# Autodesk Inventor assembly: fox
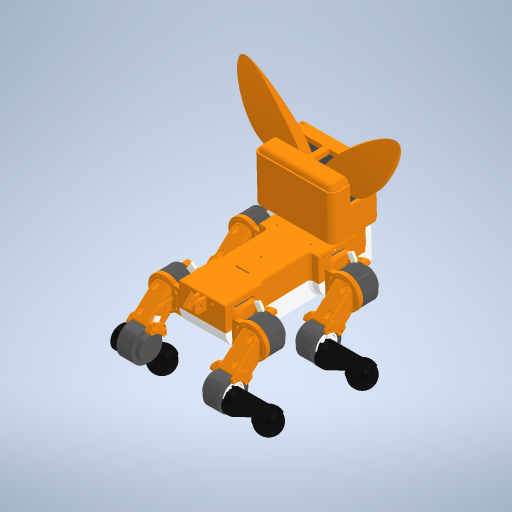
[picture p0: Inventor's stored thumbnail of the model, 512x512]
Saved by Autodesk Inventor 2024.2 (Build 282272000, 272)
## iProperties
Created: 2025-09-19
Part Number: fox
Document SubType Name: Assembly
Designer: AdminForWorker
Title: Pupper v3.5 v16
Author: AdminForWorker
## Documents named in this file (11)
- D:\dog\fox\construction\fox\fox.iam
- D:\dog\fox\construction\fox\legs\Lower leg - Short Short V6 (No Pinch) v20.iam
- D:\dog\fox\construction\fox\legs\Lower leg - Short Short V6 (No Pinch) v20_1.iam
- D:\dog\fox\construction\fox\legs\две части ног.iam
- D:\dog\fox\construction\fox\body\тело лисы.iam
- D:\dog\fox\construction\fox\legs\одна часть ноги.iam
- D:\dog\fox\construction\fox\legs\одна часть ноги симетр.iam
- D:\dog\fox\construction\fox\legs\Lower leg - Short Short V6 (No Pinch) v20(Mirror).iam
- D:\dog\fox\construction\fox\legs\Lower leg - Short Short V6 (No Pinch) v20(Mirror)_1.iam
- D:\dog\fox\construction\fox\body\аккумулятор 21700.iam
- D:\dog\fox\construction\3dstep\хвост.ipt
## Components (10 placed, 10 different names)
1. нижняя нога правая 2 [sub-assembly]
2. тело [sub-assembly] — Совмещение:1, Совмещение:2, Заподлицо:1, Совмещение:4, Цилиндрический:1, Совмещение:5, Совмещение:6, Цилиндрический:2, С поворотом:1, С поворотом:2, Заподлицо:2
3. верхняя нога левая [sub-assembly] — Цилиндрический:1, Совмещение:5, Совмещение:6
4. верхняя нога правая [sub-assembly] — Совмещение:4, Цилиндрический:2, С поворотом:1
5. нижняя нога левая 2 [sub-assembly]
6. нижняя нога левая [sub-assembly]
7. нижняя нога правая [sub-assembly]
8. верхняя нога перед [sub-assembly] — С поворотом:2
9. аккумулятор 21700:1 [sub-assembly] — Совмещение:1, Совмещение:2, Заподлицо:1
10. хвост:1 — Заподлицо:2
## Relationships (11: Mate 5, Flush 2, CylindricalJoint 2, RevoluteJoint 2)
- Совмещение:1 [Mate] (4 mm): тело ↔ аккумулятор 21700:1
- Совмещение:2 [Mate] (11 mm): тело ↔ аккумулятор 21700:1
- Заподлицо:1 [Flush]: тело ↔ аккумулятор 21700:1
- Совмещение:4 [Mate]: тело ↔ верхняя нога правая
- Цилиндрический:1 [CylindricalJoint]: тело ↔ верхняя нога левая
- Совмещение:5 [Mate]: тело ↔ верхняя нога левая
- Совмещение:6 [Mate]: тело ↔ верхняя нога левая
- Цилиндрический:2 [CylindricalJoint]: тело ↔ верхняя нога правая
- С поворотом:1 [RevoluteJoint]: тело ↔ верхняя нога правая
- С поворотом:2 [RevoluteJoint]: тело ↔ верхняя нога перед
- Заподлицо:2 [Flush]: тело ↔ хвост:1
